# Autodesk Inventor assembly: holder_assembly_2
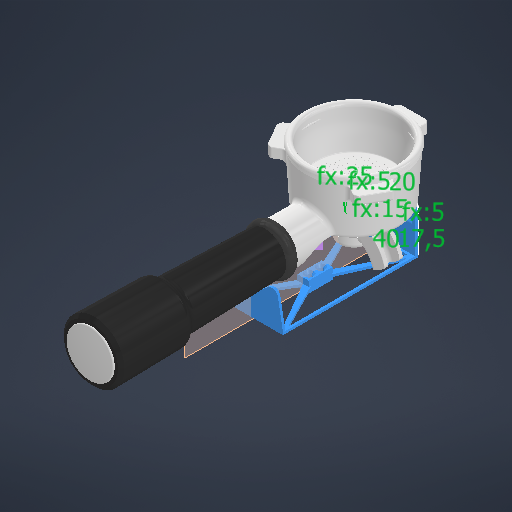
[picture p0: Inventor's stored thumbnail of the model, 512x512]
Saved by Autodesk Inventor 2026 (Build 300175000, 175)
## iProperties
Created: 2025-04-29
Part Number: holder_assembly_2
Document SubType Name: Assembly
Designer: Paul Juschitz
Author: Paul Juschitz
## Documents named in this file (3)
- C:\Users\Paul Juschitz\Documents\private\m5_GBW_mod\M5_GBW_mod\CAD\holder_assembly_2.iam
- C:\Users\Paul Juschitz\Documents\private\m5_GBW_mod\M5_GBW_mod\CAD\my_portafilter_holder_6.ipt
- C:\Users\Paul Juschitz\Documents\private\m5_GBW_mod\M5_GBW_mod\CAD\downloads\portafilter\BES870XL Portafilter\BES870XL Portafilter\BES870XL Portafilter_assembled.iam
## Components (2 placed, 2 different names)
1. my_portafilter_holder_6:1 — Mate:2
2. BES870XL Portafilter_assembled:1 [sub-assembly] — Mate:2
## Relationships (1: Mate 1)
- Mate:2: my_portafilter_holder_6:1 ↔ BES870XL Portafilter_assembled:1
